# Autodesk Inventor assembly: LED
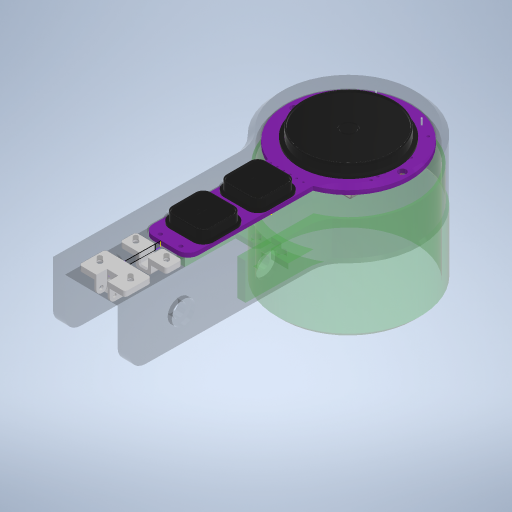
[picture p0: Inventor's stored thumbnail of the model, 512x512]
Saved by Autodesk Inventor 2024 (Build 280153000, 153)
## iProperties
Created: 2023-06-02
Part Number: LED
Document SubType Name: Assembly
Designer: lunima
Author: lunima
## Documents named in this file (10)
- C:\Users\lunima\Desktop\DOSYN\IPT\LED Cover\Dosyn LED.iam
- C:\Users\lunima\Desktop\DOSYN\IPT\LED Cover\LED Cover - Bottom.ipt
- C:\Users\lunima\Desktop\DOSYN\IPT\LED Cover\LED Cover - Top.ipt
- C:\Users\lunima\Desktop\DOSYN\IPT\Electronics\Dosyn Pad.iam
- C:\Users\lunima\Desktop\DOSYN\IPT\LED Cover\LED Cover Cable Strain Relief Clip.ipt
- C:\Users\lunima\Desktop\DOSYN\IPT\LED Cover\LED Cover Drag Chain Termination.ipt
- C:\Users\lunima\Desktop\DOSYN\IPT\Electronics\LDD-700L.ipt
- C:\Users\lunima\Desktop\DOSYN\IPT\Electronics\Seeeduino XIAO SAMD21 v4\Seeeduino XIAO SAMD21 v4.iam
- C:\Users\lunima\Desktop\DOSYN\IPT\LED Cover\Button Sockets.ipt
- C:\Users\lunima\Desktop\DOSYN\IPT\LED Cover\Buttons.ipt
## Components (9 placed, 9 different names)
1. LED Cover - Bottom:1 — 旋转:5
2. LED Cover - Top:1 — 配合:1, 平面:1, 旋转:3, 旋转:4, 旋转:5, 配合:3
3. Dosyn Pad:1 [sub-assembly] — 配合:1, 旋转:4, 旋转:6, 旋转:7
4. LED Cover Cable Strain Relief Clip:1 — 平面:1
5. LED Cover Drag Chain Termination:1 — 旋转:3
6. LDD-700L:1 — 旋转:6
7. Seeeduino XIAO SAMD21 v4:1 [sub-assembly] — 旋转:7
8. Button Sockets:1 — 配合:2, 配合:3
9. Buttons:1 — 配合:2
## Relationships (9: RevoluteJoint 5, Mate 3, PlanarJoint 1)
- 配合:1 [Mate]: LED Cover - Top:1 ↔ Dosyn Pad:1
- 平面:1 [PlanarJoint]: LED Cover - Top:1 ↔ LED Cover Cable Strain Relief Clip:1
- 旋转:3 [RevoluteJoint]: LED Cover - Top:1 ↔ LED Cover Drag Chain Termination:1
- 旋转:4 [RevoluteJoint]: LED Cover - Top:1 ↔ Dosyn Pad:1
- 旋转:5 [RevoluteJoint]: LED Cover - Bottom:1 ↔ LED Cover - Top:1
- 旋转:6 [RevoluteJoint]: Dosyn Pad:1 ↔ LDD-700L:1
- 旋转:7 [RevoluteJoint]: Dosyn Pad:1 ↔ Seeeduino XIAO SAMD21 v4:1
- 配合:2 [Mate]: Button Sockets:1 ↔ Buttons:1
- 配合:3 [Mate]: LED Cover - Top:1 ↔ Button Sockets:1
